# Autodesk Inventor assembly: 015-brs
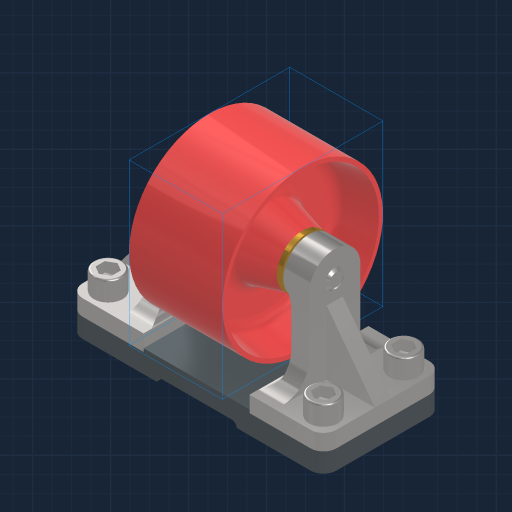
[picture p0: Inventor's stored thumbnail of the model, 512x512]
Saved by Autodesk Inventor 2024 (Build 280153000, 153)
## iProperties
Created: 2025-03-10
Part Number: 015-brs
Document SubType Name: Assembly
Designer: DuctopwH
Author: DuctopwH
## Documents named in this file (8)
- C:\Users\DuctopwH\Google Drive\projects\cadblueprints\015-РР\015-brs.iam
- C:\Users\DuctopwH\Google Drive\projects\cadblueprints\015-РР\parts\01-base.ipt
- C:\Users\DuctopwH\Google Drive\projects\cadblueprints\015-РР\parts\02-bracket.ipt
- C:\Users\DuctopwH\Google Drive\projects\cadblueprints\015-РР\parts\03-bushing.ipt
- C:\Users\DuctopwH\Google Drive\projects\cadblueprints\015-РР\parts\04-roller.ipt
- C:\Users\DuctopwH\Google Drive\projects\cadblueprints\015-РР\parts\05-spindel.ipt
- C:\Users\DuctopwH\Documents\Inventor\Content Center Files\R2024\en-US\GOST 11738-84\Screw M12-6gx20 GOST 11738-84.ipt
- C:\Users\DuctopwH\Google Drive\projects\cadblueprints\015-РР\parts\01-base_thread.ipt
## Components (12 placed, 7 different names)
1. 01-base:1 — Mate:1, Flush:1, Flush:2, Mate:2, Mate:3, Mate:4, Mate:5, Mate:6, Mate:7, Mate:15, Flush:3, Flush:4, Flush:5
2. 01-base_thread:1 — Flush:3, Flush:4, Flush:5
3. 02-bracket:1 — Mate:2, Mate:3, Mate:4, Insert:1
4. 02-bracket:2 — Mate:5, Mate:6, Mate:7, Mate:14, Insert:2
5. 03-bushing:1 — Mate:10, Mate:11
6. 03-bushing:2 — Mate:8, Mate:9, Mate:13
7. 04-roller:1 — Mate:8, Mate:9, Mate:10, Mate:11, Mate:12, Mate:15
8. 05-spindel:1 — Mate:12, Mate:13, Mate:14
9. Screw GOST 11738-84 M 12x20:1 — Insert:1
10. Screw GOST 11738-84 M 12x20:2
11. Screw GOST 11738-84 M 12x20:3 — Insert:2
12. Screw GOST 11738-84 M 12x20:4
## Component patterns: (2 elements, first: Screw GOST 11738-84 M 12x20:1), Component Pattern 2:1 (2 elements)
## Relationships (22: Mate 15, Flush 5, Insert 2)
- Mate:1: 01-base:1
- Flush:1: 01-base:1
- Flush:2: 01-base:1
- Mate:2: 01-base:1 ↔ 02-bracket:1
- Mate:3: 01-base:1 ↔ 02-bracket:1
- Mate:4: 01-base:1 ↔ 02-bracket:1
- Mate:5: 01-base:1 ↔ 02-bracket:2
- Mate:6: 01-base:1 ↔ 02-bracket:2
- Mate:7: 01-base:1 ↔ 02-bracket:2
- Mate:8: 03-bushing:2 ↔ 04-roller:1
- Mate:9: 03-bushing:2 ↔ 04-roller:1
- Mate:10: 03-bushing:1 ↔ 04-roller:1
- Mate:11: 03-bushing:1 ↔ 04-roller:1
- Mate:12: 04-roller:1 ↔ 05-spindel:1
- Mate:13: 03-bushing:2 ↔ 05-spindel:1
- Mate:14: 02-bracket:2 ↔ 05-spindel:1
- Mate:15: 01-base:1 ↔ 04-roller:1
- Insert:1: 02-bracket:1 ↔ Screw GOST 11738-84 M 12x20:1
- Insert:2: 02-bracket:2 ↔ Screw GOST 11738-84 M 12x20:3
- Flush:3: 01-base:1 ↔ 01-base_thread:1
- Flush:4: 01-base:1 ↔ 01-base_thread:1
- Flush:5: 01-base:1 ↔ 01-base_thread:1
